# Autodesk Inventor assembly: X-End-Motor v0.3
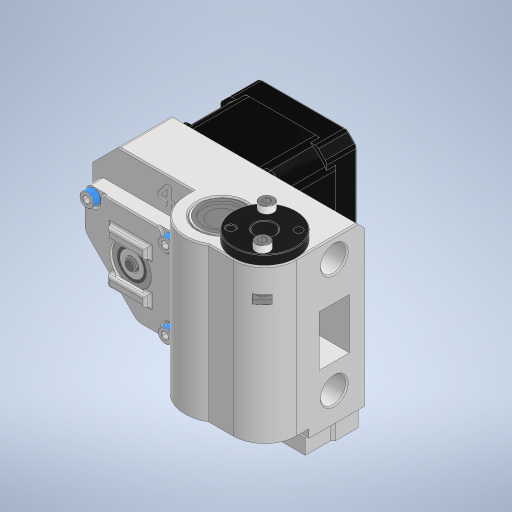
[picture p0: Inventor's stored thumbnail of the model, 512x512]
Saved by Autodesk Inventor 2023 (Build 270158000, 158)
## iProperties
Created: 2023-07-24
Part Number: X-End-Motor v0.3
Document SubType Name: Assembly
Designer: Parker
Author: Parker
## Documents named in this file (14)
- D:\000 - PEPCORP CLOUD\00- Legacy\Designs\MK3PRO P1\X-Axis\X-End-Motor v0.3.iam
- D:\000 - PEPCORP CLOUD\00- Legacy\Designs\MK3PRO P1\X-Axis\X-End-motor v0.3.ipt
- X-End-motor v0.4.ipt
- D:\000 - PEPCORP CLOUD\00- Legacy\Designs\MK3PRO P1\X-Axis\Teflon T-Nut.ipt
- D:\000 - PEPCORP CLOUD\00- Legacy\Designs\MK3PRO P1\X-Axis\x-axis-stepper-motor.iam
- D:\000 - PEPCORP CLOUD\00- Legacy\Designs\MK3PRO P1\COMPONENTS\625 Bearing.ipt
- D:\000 - PEPCORP CLOUD\00- Legacy\Designs\MK3PRO P1\COMPONENTS\LM10UU.ipt
- D:\000 - PEPCORP CLOUD\00- Legacy\Designs\MK3PRO P1\COMPONENTS\GT2_16T.ipt
- D:\000 - PEPCORP CLOUD\00- Legacy\Designs\MK3PRO P1\COMPONENTS\Small Limit Switch.iam
- D:\000 - PEPCORP CLOUD\00- Legacy\Designs\MK3PRO P1\COMPONENTS\SHCS_M2_10.ipt
- D:\000 - PEPCORP CLOUD\00- Legacy\Designs\MK3PRO P1\COMPONENTS\SHCS_M3_18.ipt
- D:\000 - PEPCORP CLOUD\00- Legacy\Designs\MK3PRO P1\COMPONENTS\NUT_SQUARE_M3.ipt
- D:\000 - PEPCORP CLOUD\00- Legacy\Designs\MK3PRO P1\X-Axis\X-Axis-Motor-Support v0.1.ipt
- D:\000 - PEPCORP CLOUD\00- Legacy\Designs\MK3PRO P1\COMPONENTS\SHCS_M3_30.ipt
## Components (18 placed, 12 different names)
1. X-End-motor v0.4:1 — Flush:1, Flush:2, Flush:3, Mate:1, Mate:2, Mate:5, Flush:5, Mate:6, Mate:8, Mate:9, Mate:12, Mate:13, Mate:14, Mate:19, Mate:20, Mate:21, Angle:1, Mate:24, Angle:2, Mate:25, Mate:28, Mate:29, Mate:30
2. Teflon T-Nut:1 — Mate:8, Mate:9, Mate:21, Mate:22, Mate:23, Mate:26, Mate:27
3. x-axis-stepper-motor:1 [sub-assembly] — Mate:1, Mate:2, Mate:10, Mate:11, Mate:38
4. 625 Bearing:1 — Mate:31, Mate:39
5. LM10UU:1 — Mate:6, Mate:7
6. LM10UU:2 — Mate:5, Flush:5, Mate:7
7. GT2_16T:1 — Mate:10, Mate:11, Mate:31
8. Small Limit Switch:1 [sub-assembly] — Mate:12, Mate:13, Mate:14, Mate:15, Mate:16, Mate:17, Mate:18
9. SHCS_M2_10:1 — Mate:16, Mate:17
10. SHCS_M2_10:2 — Mate:15, Mate:18
11. SHCS_M3_18:1 — Mate:22, Mate:23
12. SHCS_M3_18:2 — Mate:26, Mate:27
13. NUT_SQUARE_M3:1 — Mate:19, Mate:20, Angle:1
14. NUT_SQUARE_M3:2 — Mate:24, Angle:2, Mate:25
15. X-Axis-Motor-Support v0.1:1 — Mate:28, Mate:29, Mate:30, Mate:32, Mate:33, Mate:34, Mate:35, Mate:36, Mate:37, Mate:39
16. SHCS_M3_30:1 — Mate:32, Mate:36
17. SHCS_M3_30:2 — Mate:33, Mate:37
18. SHCS_M3_30:3 — Mate:34, Mate:35, Mate:38
## Relationships (43: Mate 37, Flush 4, Angle 2)
- Flush:1: X-End-motor v0.4:1
- Flush:2: X-End-motor v0.4:1
- Flush:3: X-End-motor v0.4:1
- Mate:1: X-End-motor v0.4:1 ↔ x-axis-stepper-motor:1
- Mate:2: X-End-motor v0.4:1 ↔ x-axis-stepper-motor:1
- Mate:5: X-End-motor v0.4:1 ↔ LM10UU:2
- Flush:5: X-End-motor v0.4:1 ↔ LM10UU:2
- Mate:6: X-End-motor v0.4:1 ↔ LM10UU:1
- Mate:7: LM10UU:1 ↔ LM10UU:2
- Mate:8: X-End-motor v0.4:1 ↔ Teflon T-Nut:1
- Mate:9: X-End-motor v0.4:1 ↔ Teflon T-Nut:1
- Mate:10 (0.5 mm): x-axis-stepper-motor:1 ↔ GT2_16T:1
- Mate:11: x-axis-stepper-motor:1 ↔ GT2_16T:1
- Mate:12: X-End-motor v0.4:1 ↔ Small Limit Switch:1
- Mate:13: X-End-motor v0.4:1 ↔ Small Limit Switch:1
- Mate:14: X-End-motor v0.4:1 ↔ Small Limit Switch:1
- Mate:15: Small Limit Switch:1 ↔ SHCS_M2_10:2
- Mate:16: Small Limit Switch:1 ↔ SHCS_M2_10:1
- Mate:17: Small Limit Switch:1 ↔ SHCS_M2_10:1
- Mate:18: Small Limit Switch:1 ↔ SHCS_M2_10:2
- Mate:19: X-End-motor v0.4:1 ↔ NUT_SQUARE_M3:1
- Mate:20: X-End-motor v0.4:1 ↔ NUT_SQUARE_M3:1
- Mate:21: X-End-motor v0.4:1 ↔ Teflon T-Nut:1
- Angle:1 (0 deg): X-End-motor v0.4:1 ↔ NUT_SQUARE_M3:1
- Mate:22: Teflon T-Nut:1 ↔ SHCS_M3_18:1
- Mate:23: Teflon T-Nut:1 ↔ SHCS_M3_18:1
- Mate:24: X-End-motor v0.4:1 ↔ NUT_SQUARE_M3:2
- Angle:2 (0 deg): X-End-motor v0.4:1 ↔ NUT_SQUARE_M3:2
- Mate:25: X-End-motor v0.4:1 ↔ NUT_SQUARE_M3:2
- Mate:26: Teflon T-Nut:1 ↔ SHCS_M3_18:2
- Mate:27: Teflon T-Nut:1 ↔ SHCS_M3_18:2
- Mate:28: X-End-motor v0.4:1 ↔ X-Axis-Motor-Support v0.1:1
- Mate:29: X-End-motor v0.4:1 ↔ X-Axis-Motor-Support v0.1:1
- Mate:30: X-End-motor v0.4:1 ↔ X-Axis-Motor-Support v0.1:1
- Mate:31 (1 mm): 625 Bearing:1 ↔ GT2_16T:1
- Mate:32: X-Axis-Motor-Support v0.1:1 ↔ SHCS_M3_30:1
- Mate:33: X-Axis-Motor-Support v0.1:1 ↔ SHCS_M3_30:2
- Mate:34: X-Axis-Motor-Support v0.1:1 ↔ SHCS_M3_30:3
- Mate:35: X-Axis-Motor-Support v0.1:1 ↔ SHCS_M3_30:3
- Mate:36: X-Axis-Motor-Support v0.1:1 ↔ SHCS_M3_30:1
- Mate:37: X-Axis-Motor-Support v0.1:1 ↔ SHCS_M3_30:2
- Mate:38: x-axis-stepper-motor:1 ↔ SHCS_M3_30:3
- Mate:39: 625 Bearing:1 ↔ X-Axis-Motor-Support v0.1:1
